# Autodesk Inventor assembly: FE-00036LowerFrame_MIR
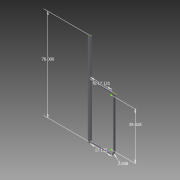
[picture p0: Inventor's stored thumbnail of the model, 180x180]
Saved by Autodesk Inventor 2013 (Build 170138000, 138)
## iProperties
Created: 2013-01-13
Part Number: FE-00036LowerFrame_MIR
Document SubType Name: Assembly
Designer: Phillip
Author: Phillip
## Documents named in this file (5)
- C:\Users\Moses\Documents\Inventor\2013 Team 3061 Robot\FIRST Arena 2013\Feeder Goal Station\FE-00036LowerFrame_MIR.iam
- C:\Users\Moses\Documents\Inventor\2013 Team 3061 Robot\FIRST Arena 2013\Feeder Goal Station\FE00036LowerFrame_MIR.ipt
- C:\Users\Moses\Documents\Inventor\2013 Team 3061 Robot\FIRST Arena 2013\Feeder Goal Station\FE-00036LowerFrame\Frame\Frame0001_MIR.iam
- C:\Users\Moses\Documents\Inventor\2013 Team 3061 Robot\FIRST Arena 2013\Feeder Goal Station\Frame0002_MIR.ipt
- C:\Users\Moses\Documents\Inventor\2013 Team 3061 Robot\FIRST Arena 2013\Feeder Goal Station\FE-00036Base_MIR.ipt
## Components (4 placed, 4 different names)
1. FE00036LowerFrame_MIR:1
2. Frame0001_MIR:1 [sub-assembly] — Mate:1
3. Frame0002_MIR:1 — Flush:1, Flush:2
4. FE-00036Base_MIR:1 — Flush:2
## Relationships (3: Mate 3)
- Flush:1 [Mate]: Frame0002_MIR:1
- Flush:2 [Mate]: Frame0002_MIR:1 ↔ FE-00036Base_MIR:1
- Mate:1: Frame0001_MIR:1
